# Autodesk Inventor assembly: CNC-1.1v-XA-1
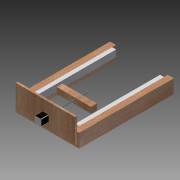
[picture p0: Inventor's stored thumbnail of the model, 180x180]
Saved by Autodesk Inventor 2015 (Build 190159000, 159)
## iProperties
Created: 2015-07-10
Part Number: CNC-1.1v-XA-1
Document SubType Name: Assembly
Designer: Bangladesh
Author: Bangladesh
## Documents named in this file (8)
- C:\Users\Alvi\Documents\CNC design files\CNC_1.1v\CNC-1.1v-XA-1.iam
- C:\Users\Alvi\Documents\CNC design files\CNC_1.1v\CNC-1.1v-X-2-(main 2 by 4).ipt
- C:\Users\Alvi\Documents\CNC design files\CNC_1.1v\CNC-1.1v-X-3-(lineardrawer).ipt
- C:\Users\Alvi\Documents\CNC design files\CNC_1.1v\CNC-1.1v-X-1-(faceplate).ipt
- C:\Users\Alvi\Documents\CNC design files\CNC_1.1v\CNC-1.1v-X-7-( short thread rod).ipt
- C:\Users\Alvi\Documents\CNC design files\CNC_1.1v\CNC-1.1v-XP-1-(face plate).iam
- C:\Users\Alvi\Documents\CNC design files\CNC_1.1v\CNC-1.1v-B-2-( circular nut ).ipt
- C:\Users\Alvi\Documents\CNC design files\CNC_1.1v\CNC-1.1v-X-8-( axis mover nut inside).ipt
## Components (9 placed, 7 different names)
1. CNC-1.1v-X-1-(faceplate):1 — Mate:33, Mate:36, Mate:37, Mate:38, Mate:39, Mate:40, Mate:41, Mate:42, Mate:44, Mate:45, Mate:49, Mate:50
2. CNC-1.1v-X-7-( short thread rod):1 — Mate:34, Mate:35, Mate:48
3. CNC-1.1v-XP-1-(face plate):1 [sub-assembly] — Mate:33, Mate:34, Mate:35, Mate:49, Mate:50
4. CNC-1.1v-X-2-(main 2 by 4):1 — Mate:39, Mate:40, Mate:41, Mate:46, Mate:47
5. CNC-1.1v-X-2-(main 2 by 4):2 — Mate:36, Mate:37, Mate:38, Mate:43
6. CNC-1.1v-X-3-(lineardrawer):1 — Mate:42, Mate:43, Mate:44
7. CNC-1.1v-X-3-(lineardrawer):2 — Mate:45, Mate:46, Mate:47
8. CNC-1.1v-B-2-( circular nut ):1 — Mate:48, Flush:1, Mate:51
9. CNC-1.1v-X-8-( axis mover nut inside):1 — Flush:1, Mate:51
## Relationships (20: Mate 19, Flush 1)
- Mate:33: CNC-1.1v-X-1-(faceplate):1 ↔ CNC-1.1v-XP-1-(face plate):1
- Mate:34: CNC-1.1v-X-7-( short thread rod):1 ↔ CNC-1.1v-XP-1-(face plate):1
- Mate:35: CNC-1.1v-X-7-( short thread rod):1 ↔ CNC-1.1v-XP-1-(face plate):1
- Mate:36: CNC-1.1v-X-1-(faceplate):1 ↔ CNC-1.1v-X-2-(main 2 by 4):2
- Mate:37: CNC-1.1v-X-1-(faceplate):1 ↔ CNC-1.1v-X-2-(main 2 by 4):2
- Mate:38: CNC-1.1v-X-1-(faceplate):1 ↔ CNC-1.1v-X-2-(main 2 by 4):2
- Mate:39: CNC-1.1v-X-1-(faceplate):1 ↔ CNC-1.1v-X-2-(main 2 by 4):1
- Mate:40: CNC-1.1v-X-1-(faceplate):1 ↔ CNC-1.1v-X-2-(main 2 by 4):1
- Mate:41: CNC-1.1v-X-1-(faceplate):1 ↔ CNC-1.1v-X-2-(main 2 by 4):1
- Mate:42: CNC-1.1v-X-1-(faceplate):1 ↔ CNC-1.1v-X-3-(lineardrawer):1
- Mate:43: CNC-1.1v-X-2-(main 2 by 4):2 ↔ CNC-1.1v-X-3-(lineardrawer):1
- Mate:44: CNC-1.1v-X-1-(faceplate):1 ↔ CNC-1.1v-X-3-(lineardrawer):1
- Mate:45: CNC-1.1v-X-1-(faceplate):1 ↔ CNC-1.1v-X-3-(lineardrawer):2
- Mate:46: CNC-1.1v-X-2-(main 2 by 4):1 ↔ CNC-1.1v-X-3-(lineardrawer):2
- Mate:47: CNC-1.1v-X-2-(main 2 by 4):1 ↔ CNC-1.1v-X-3-(lineardrawer):2
- Mate:48: CNC-1.1v-X-7-( short thread rod):1 ↔ CNC-1.1v-B-2-( circular nut ):1
- Mate:49 (14 mm): CNC-1.1v-X-1-(faceplate):1 ↔ CNC-1.1v-XP-1-(face plate):1
- Mate:50 (24 mm): CNC-1.1v-X-1-(faceplate):1 ↔ CNC-1.1v-XP-1-(face plate):1
- Flush:1: CNC-1.1v-B-2-( circular nut ):1 ↔ CNC-1.1v-X-8-( axis mover nut inside):1
- Mate:51: CNC-1.1v-B-2-( circular nut ):1 ↔ CNC-1.1v-X-8-( axis mover nut inside):1
